# Autodesk Inventor assembly: fullbox
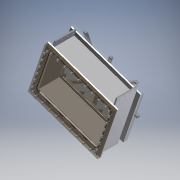
[picture p0: Inventor's stored thumbnail of the model, 180x180]
Saved by Autodesk Inventor 2017 (Build 210142000, 142)
## iProperties
Created: 2017-08-02
Part Number: fullbox
Document SubType Name: Assembly
Designer: Kai
Author: Kai
## Documents named in this file (14)
- D:\robosub\fullbox.iam
- C:\Users\Kai\Documents\Sub_stuff\2018sub\box2.0\longsides.ipt
- C:\Users\Kai\Documents\Sub_stuff\2018sub\box2.0\shortsides.ipt
- C:\Users\Kai\Documents\Sub_stuff\2018sub\box2.0\smallgasketback.ipt
- C:\Users\Kai\Downloads\91292A137_TYPE 18-8 SS SOCKET HEAD CAP SCREW.ipt
- C:\Users\Kai\Documents\Sub_stuff\2018sub\box2.0\top.ipt
- C:\Users\Kai\Documents\Sub_stuff\2018sub\box2.0\toppoly.ipt
- C:\Users\Kai\Documents\Sub_stuff\2018sub\box2.0\bottom3.ipt
- C:\Users\Kai\Documents\Sub_stuff\2018sub\box2.0\alumbottom3.ipt
- C:\Users\Kai\Documents\Sub_stuff\2018sub\box2.0\lock\pin holder.ipt
- C:\Users\Kai\Documents\Sub_stuff\2018sub\box2.0\lock\pins.ipt
- C:\Users\Kai\Downloads\91292A134_TYPE 18-8 SS SOCKET HEAD CAP SCREW.ipt
- C:\Users\Kai\Documents\Sub_stuff\2018sub\box2.0\lid guide.ipt
- C:\Users\Kai\Downloads\99397A074_METRIC THREAD-FORMING SCREW FOR PLASTICS.ipt
## Components (65 placed, 13 different names)
1. longsides:1 — Mate:6, Flush:8
2. longsides:2 — Mate:3, Mate:106, Mate:107, Mate:108, Mate:109, Flush:3
3. shortsides:1 — Mate:3, Mate:106, Mate:108, Flush:9, Mate:116
4. shortsides:2 — Mate:6, Mate:107, Mate:109, Mate:111, Mate:112
5. smallgasketback:1 — Mate:117, Mate:118
6. top:1 — Mate:111, Mate:112, Flush:3, Mate:113, Mate:114, Mate:115, Flush:4, Flush:5, Mate:213, Mate:214
7. smallgasketback:2 — Mate:113, Mate:114
8. toppoly:1 — Mate:115, Flush:4, Flush:5, Mate:193, Flush:10, Flush:11, Mate:212
9. bottom3:1 — Mate:119, Mate:120, Mate:121, Mate:122, Mate:123, Mate:124, Mate:125, Mate:126, Mate:127, Mate:128, Mate:129, Mate:130, Mate:131, Mate:132, Mate:133, Mate:134, Mate:135, Mate:136, Mate:137, Mate:138, Mate:139, Mate:140, Mate:141, Mate:142, Mate:143, Mate:144, Mate:145, Mate:146, Mate:147, Mate:148, Mate:149, Mate:150, Mate:151, Mate:152, Mate:153, Mate:154, Mate:155, Mate:156, Mate:157, Mate:158, Mate:159, Mate:160, Mate:161, Mate:162, Mate:163, Mate:164, Mate:165, Mate:166, Mate:167, Mate:168, Mate:169, Mate:170, Mate:171, Mate:172, Mate:173, Mate:174, Mate:175, Mate:176, Mate:177, Mate:178, Mate:179, Mate:180, Mate:181, Mate:182, Mate:183, Mate:184, Mate:185, Mate:186, Mate:187, Mate:188, Mate:189
10. alumbottom3:1 — Flush:8, Flush:9, Mate:116, Mate:117, Mate:118, Mate:119, Mate:120, Mate:121
11. 91292A137_TYPE 18-8 SS SOCKET HEAD CAP SCREW:1 — Mate:123, Mate:188
12. 91292A137_TYPE 18-8 SS SOCKET HEAD CAP SCREW:2 — Mate:124, Mate:189
13. 91292A137_TYPE 18-8 SS SOCKET HEAD CAP SCREW:3 — Mate:125, Mate:158
14. 91292A137_TYPE 18-8 SS SOCKET HEAD CAP SCREW:4 — Mate:126, Mate:157
15. 91292A137_TYPE 18-8 SS SOCKET HEAD CAP SCREW:5 — Mate:127, Mate:156
16. 91292A137_TYPE 18-8 SS SOCKET HEAD CAP SCREW:6 — Mate:128, Mate:159
17. 91292A137_TYPE 18-8 SS SOCKET HEAD CAP SCREW:7 — Mate:129, Mate:160
18. 91292A137_TYPE 18-8 SS SOCKET HEAD CAP SCREW:8 — Mate:130, Mate:161
19. 91292A137_TYPE 18-8 SS SOCKET HEAD CAP SCREW:9 — Mate:131, Mate:162
20. 91292A137_TYPE 18-8 SS SOCKET HEAD CAP SCREW:10 — Mate:132, Mate:163
21. 91292A137_TYPE 18-8 SS SOCKET HEAD CAP SCREW:11 — Mate:133, Mate:164
22. 91292A137_TYPE 18-8 SS SOCKET HEAD CAP SCREW:12 — Mate:134, Mate:165
23. 91292A137_TYPE 18-8 SS SOCKET HEAD CAP SCREW:13 — Mate:135, Mate:166
24. 91292A137_TYPE 18-8 SS SOCKET HEAD CAP SCREW:14 — Mate:136, Mate:167
25. 91292A137_TYPE 18-8 SS SOCKET HEAD CAP SCREW:15 — Mate:137, Mate:168
26. 91292A137_TYPE 18-8 SS SOCKET HEAD CAP SCREW:16 — Mate:138, Mate:169
27. 91292A137_TYPE 18-8 SS SOCKET HEAD CAP SCREW:17 — Mate:139, Mate:170
28. 91292A137_TYPE 18-8 SS SOCKET HEAD CAP SCREW:18 — Mate:140, Mate:171
29. 91292A137_TYPE 18-8 SS SOCKET HEAD CAP SCREW:19 — Mate:141, Mate:172
30. 91292A137_TYPE 18-8 SS SOCKET HEAD CAP SCREW:20 — Mate:142, Mate:173
31. 91292A137_TYPE 18-8 SS SOCKET HEAD CAP SCREW:21 — Mate:144, Mate:175
32. 91292A137_TYPE 18-8 SS SOCKET HEAD CAP SCREW:22 — Mate:143, Mate:174
33. 91292A137_TYPE 18-8 SS SOCKET HEAD CAP SCREW:23 — Mate:145, Mate:176
34. 91292A137_TYPE 18-8 SS SOCKET HEAD CAP SCREW:24 — Mate:147, Mate:178
35. 91292A137_TYPE 18-8 SS SOCKET HEAD CAP SCREW:25 — Mate:148, Mate:179
36. 91292A137_TYPE 18-8 SS SOCKET HEAD CAP SCREW:26 — Mate:149, Mate:180
37. 91292A137_TYPE 18-8 SS SOCKET HEAD CAP SCREW:27 — Mate:150, Mate:181
38. 91292A137_TYPE 18-8 SS SOCKET HEAD CAP SCREW:28 — Mate:151, Mate:182
39. 91292A137_TYPE 18-8 SS SOCKET HEAD CAP SCREW:29 — Mate:152, Mate:183
40. 91292A137_TYPE 18-8 SS SOCKET HEAD CAP SCREW:30 — Mate:153, Mate:184
41. 91292A137_TYPE 18-8 SS SOCKET HEAD CAP SCREW:31 — Mate:154, Mate:185
42. 91292A137_TYPE 18-8 SS SOCKET HEAD CAP SCREW:32 — Mate:155, Mate:186
43. 91292A137_TYPE 18-8 SS SOCKET HEAD CAP SCREW:33 — Mate:146, Mate:177
44. 91292A137_TYPE 18-8 SS SOCKET HEAD CAP SCREW:34 — Mate:122, Mate:187
45. pin holder:1 — Mate:194, Mate:195
46. pins:1 — Mate:193, Mate:194, Mate:195, Flush:10, Flush:11, Mate:196, Mate:197, Mate:198, Mate:199, Mate:200, Mate:201, Mate:202, Mate:203, Mate:204, Mate:205, Mate:206, Mate:207, Mate:208, Mate:209, Mate:210, Mate:211
47. 91292A134_TYPE 18-8 SS SOCKET HEAD CAP SCREW:1 — Mate:199, Mate:208
48. 91292A134_TYPE 18-8 SS SOCKET HEAD CAP SCREW:2 — Mate:201, Mate:205
49. 91292A134_TYPE 18-8 SS SOCKET HEAD CAP SCREW:3 — Mate:200, Mate:207
50. 91292A134_TYPE 18-8 SS SOCKET HEAD CAP SCREW:4 — Mate:202, Mate:211
51. 91292A134_TYPE 18-8 SS SOCKET HEAD CAP SCREW:5 — Mate:197, Mate:209
52. 91292A134_TYPE 18-8 SS SOCKET HEAD CAP SCREW:6 — Mate:196, Mate:204
53. 91292A134_TYPE 18-8 SS SOCKET HEAD CAP SCREW:7 — Mate:198, Mate:210
54. 91292A134_TYPE 18-8 SS SOCKET HEAD CAP SCREW:8 — Mate:203, Mate:206
55. lid guide:1 — Mate:212, Mate:213, Mate:214, Mate:215, Mate:216, Mate:217, Mate:218, Mate:219, Mate:220, Mate:221, Mate:222, Mate:223, Mate:224, Mate:225, Mate:226, Mate:227, Mate:228, Mate:229, Mate:230, Mate:231, Mate:232, Mate:233, Mate:234
56. 99397A074_METRIC THREAD-FORMING SCREW FOR PLASTICS:1 — Mate:224, Mate:226
57. 99397A074_METRIC THREAD-FORMING SCREW FOR PLASTICS:2 — Mate:215, Mate:231
58. 99397A074_METRIC THREAD-FORMING SCREW FOR PLASTICS:3 — Mate:221, Mate:228
59. 99397A074_METRIC THREAD-FORMING SCREW FOR PLASTICS:4 — Mate:222, Mate:227
60. 99397A074_METRIC THREAD-FORMING SCREW FOR PLASTICS:5 — Mate:217, Mate:230
61. 99397A074_METRIC THREAD-FORMING SCREW FOR PLASTICS:6 — Mate:216, Mate:232
62. 99397A074_METRIC THREAD-FORMING SCREW FOR PLASTICS:7 — Mate:223, Mate:225
63. 99397A074_METRIC THREAD-FORMING SCREW FOR PLASTICS:8 — Mate:219, Mate:229
64. 99397A074_METRIC THREAD-FORMING SCREW FOR PLASTICS:9 — Mate:218, Mate:233
65. 99397A074_METRIC THREAD-FORMING SCREW FOR PLASTICS:10 — Mate:220, Mate:234
## Relationships (134: Mate 127, Flush 7)
- Mate:3: longsides:2 ↔ shortsides:1
- Mate:6: longsides:1 ↔ shortsides:2
- Mate:106: longsides:2 ↔ shortsides:1
- Mate:107: longsides:2 ↔ shortsides:2
- Mate:108: longsides:2 ↔ shortsides:1
- Mate:109: longsides:2 ↔ shortsides:2
- Mate:111: shortsides:2 ↔ top:1
- Mate:112 (304.8 mm): shortsides:2 ↔ top:1
- Flush:3 (-19.05 mm): longsides:2 ↔ top:1
- Mate:113: top:1 ↔ smallgasketback:2
- Mate:114: top:1 ↔ smallgasketback:2
- Mate:115: top:1 ↔ toppoly:1
- Flush:4: top:1 ↔ toppoly:1
- Flush:5: top:1 ↔ toppoly:1
- Flush:8: longsides:1 ↔ alumbottom3:1
- Flush:9: shortsides:1 ↔ alumbottom3:1
- Mate:116: shortsides:1 ↔ alumbottom3:1
- Mate:117: smallgasketback:1 ↔ alumbottom3:1
- Mate:118: smallgasketback:1 ↔ alumbottom3:1
- Mate:119: bottom3:1 ↔ alumbottom3:1
- Mate:120: bottom3:1 ↔ alumbottom3:1
- Mate:121: bottom3:1 ↔ alumbottom3:1
- Mate:122: bottom3:1 ↔ 91292A137_TYPE 18-8 SS SOCKET HEAD CAP SCREW:34
- Mate:123: bottom3:1 ↔ 91292A137_TYPE 18-8 SS SOCKET HEAD CAP SCREW:1
- Mate:124: bottom3:1 ↔ 91292A137_TYPE 18-8 SS SOCKET HEAD CAP SCREW:2
- Mate:125: bottom3:1 ↔ 91292A137_TYPE 18-8 SS SOCKET HEAD CAP SCREW:3
- Mate:126: bottom3:1 ↔ 91292A137_TYPE 18-8 SS SOCKET HEAD CAP SCREW:4
- Mate:127: bottom3:1 ↔ 91292A137_TYPE 18-8 SS SOCKET HEAD CAP SCREW:5
- Mate:128: bottom3:1 ↔ 91292A137_TYPE 18-8 SS SOCKET HEAD CAP SCREW:6
- Mate:129: bottom3:1 ↔ 91292A137_TYPE 18-8 SS SOCKET HEAD CAP SCREW:7
- Mate:130: bottom3:1 ↔ 91292A137_TYPE 18-8 SS SOCKET HEAD CAP SCREW:8
- Mate:131: bottom3:1 ↔ 91292A137_TYPE 18-8 SS SOCKET HEAD CAP SCREW:9
- Mate:132: bottom3:1 ↔ 91292A137_TYPE 18-8 SS SOCKET HEAD CAP SCREW:10
- Mate:133: bottom3:1 ↔ 91292A137_TYPE 18-8 SS SOCKET HEAD CAP SCREW:11
- Mate:134: bottom3:1 ↔ 91292A137_TYPE 18-8 SS SOCKET HEAD CAP SCREW:12
- Mate:135: bottom3:1 ↔ 91292A137_TYPE 18-8 SS SOCKET HEAD CAP SCREW:13
- Mate:136: bottom3:1 ↔ 91292A137_TYPE 18-8 SS SOCKET HEAD CAP SCREW:14
- Mate:137: bottom3:1 ↔ 91292A137_TYPE 18-8 SS SOCKET HEAD CAP SCREW:15
- Mate:138: bottom3:1 ↔ 91292A137_TYPE 18-8 SS SOCKET HEAD CAP SCREW:16
- Mate:139: bottom3:1 ↔ 91292A137_TYPE 18-8 SS SOCKET HEAD CAP SCREW:17
- Mate:140: bottom3:1 ↔ 91292A137_TYPE 18-8 SS SOCKET HEAD CAP SCREW:18
- Mate:141: bottom3:1 ↔ 91292A137_TYPE 18-8 SS SOCKET HEAD CAP SCREW:19
- Mate:142: bottom3:1 ↔ 91292A137_TYPE 18-8 SS SOCKET HEAD CAP SCREW:20
- Mate:143: bottom3:1 ↔ 91292A137_TYPE 18-8 SS SOCKET HEAD CAP SCREW:22
- Mate:144: bottom3:1 ↔ 91292A137_TYPE 18-8 SS SOCKET HEAD CAP SCREW:21
- Mate:145: bottom3:1 ↔ 91292A137_TYPE 18-8 SS SOCKET HEAD CAP SCREW:23
- Mate:146: bottom3:1 ↔ 91292A137_TYPE 18-8 SS SOCKET HEAD CAP SCREW:33
- Mate:147: bottom3:1 ↔ 91292A137_TYPE 18-8 SS SOCKET HEAD CAP SCREW:24
- Mate:148: bottom3:1 ↔ 91292A137_TYPE 18-8 SS SOCKET HEAD CAP SCREW:25
- Mate:149: bottom3:1 ↔ 91292A137_TYPE 18-8 SS SOCKET HEAD CAP SCREW:26
- Mate:150: bottom3:1 ↔ 91292A137_TYPE 18-8 SS SOCKET HEAD CAP SCREW:27
- Mate:151: bottom3:1 ↔ 91292A137_TYPE 18-8 SS SOCKET HEAD CAP SCREW:28
- Mate:152: bottom3:1 ↔ 91292A137_TYPE 18-8 SS SOCKET HEAD CAP SCREW:29
- Mate:153: bottom3:1 ↔ 91292A137_TYPE 18-8 SS SOCKET HEAD CAP SCREW:30
- Mate:154: bottom3:1 ↔ 91292A137_TYPE 18-8 SS SOCKET HEAD CAP SCREW:31
- Mate:155: bottom3:1 ↔ 91292A137_TYPE 18-8 SS SOCKET HEAD CAP SCREW:32
- Mate:156: bottom3:1 ↔ 91292A137_TYPE 18-8 SS SOCKET HEAD CAP SCREW:5
- Mate:157: bottom3:1 ↔ 91292A137_TYPE 18-8 SS SOCKET HEAD CAP SCREW:4
- Mate:158: bottom3:1 ↔ 91292A137_TYPE 18-8 SS SOCKET HEAD CAP SCREW:3
- Mate:159: bottom3:1 ↔ 91292A137_TYPE 18-8 SS SOCKET HEAD CAP SCREW:6
- Mate:160: bottom3:1 ↔ 91292A137_TYPE 18-8 SS SOCKET HEAD CAP SCREW:7
- Mate:161: bottom3:1 ↔ 91292A137_TYPE 18-8 SS SOCKET HEAD CAP SCREW:8
- Mate:162: bottom3:1 ↔ 91292A137_TYPE 18-8 SS SOCKET HEAD CAP SCREW:9
- Mate:163: bottom3:1 ↔ 91292A137_TYPE 18-8 SS SOCKET HEAD CAP SCREW:10
- Mate:164: bottom3:1 ↔ 91292A137_TYPE 18-8 SS SOCKET HEAD CAP SCREW:11
- Mate:165: bottom3:1 ↔ 91292A137_TYPE 18-8 SS SOCKET HEAD CAP SCREW:12
- Mate:166: bottom3:1 ↔ 91292A137_TYPE 18-8 SS SOCKET HEAD CAP SCREW:13
- Mate:167: bottom3:1 ↔ 91292A137_TYPE 18-8 SS SOCKET HEAD CAP SCREW:14
- Mate:168: bottom3:1 ↔ 91292A137_TYPE 18-8 SS SOCKET HEAD CAP SCREW:15
- Mate:169: bottom3:1 ↔ 91292A137_TYPE 18-8 SS SOCKET HEAD CAP SCREW:16
- Mate:170: bottom3:1 ↔ 91292A137_TYPE 18-8 SS SOCKET HEAD CAP SCREW:17
- Mate:171: bottom3:1 ↔ 91292A137_TYPE 18-8 SS SOCKET HEAD CAP SCREW:18
- Mate:172: bottom3:1 ↔ 91292A137_TYPE 18-8 SS SOCKET HEAD CAP SCREW:19
- Mate:173: bottom3:1 ↔ 91292A137_TYPE 18-8 SS SOCKET HEAD CAP SCREW:20
- Mate:174: bottom3:1 ↔ 91292A137_TYPE 18-8 SS SOCKET HEAD CAP SCREW:22
- Mate:175: bottom3:1 ↔ 91292A137_TYPE 18-8 SS SOCKET HEAD CAP SCREW:21
- Mate:176: bottom3:1 ↔ 91292A137_TYPE 18-8 SS SOCKET HEAD CAP SCREW:23
- Mate:177: bottom3:1 ↔ 91292A137_TYPE 18-8 SS SOCKET HEAD CAP SCREW:33
- Mate:178: bottom3:1 ↔ 91292A137_TYPE 18-8 SS SOCKET HEAD CAP SCREW:24
- Mate:179: bottom3:1 ↔ 91292A137_TYPE 18-8 SS SOCKET HEAD CAP SCREW:25
- Mate:180: bottom3:1 ↔ 91292A137_TYPE 18-8 SS SOCKET HEAD CAP SCREW:26
- Mate:181: bottom3:1 ↔ 91292A137_TYPE 18-8 SS SOCKET HEAD CAP SCREW:27
- Mate:182: bottom3:1 ↔ 91292A137_TYPE 18-8 SS SOCKET HEAD CAP SCREW:28
- Mate:183: bottom3:1 ↔ 91292A137_TYPE 18-8 SS SOCKET HEAD CAP SCREW:29
- Mate:184: bottom3:1 ↔ 91292A137_TYPE 18-8 SS SOCKET HEAD CAP SCREW:30
- Mate:185: bottom3:1 ↔ 91292A137_TYPE 18-8 SS SOCKET HEAD CAP SCREW:31
- Mate:186: bottom3:1 ↔ 91292A137_TYPE 18-8 SS SOCKET HEAD CAP SCREW:32
- Mate:187: bottom3:1 ↔ 91292A137_TYPE 18-8 SS SOCKET HEAD CAP SCREW:34
- Mate:188: bottom3:1 ↔ 91292A137_TYPE 18-8 SS SOCKET HEAD CAP SCREW:1
- Mate:189: bottom3:1 ↔ 91292A137_TYPE 18-8 SS SOCKET HEAD CAP SCREW:2
- Mate:193: toppoly:1 ↔ pins:1
- Mate:194: pin holder:1 ↔ pins:1
- Mate:195: pin holder:1 ↔ pins:1
- Flush:10 (-6.35 mm): toppoly:1 ↔ pins:1
- Flush:11 (-6.35 mm): toppoly:1 ↔ pins:1
- Mate:196: pins:1 ↔ 91292A134_TYPE 18-8 SS SOCKET HEAD CAP SCREW:6
- Mate:197: pins:1 ↔ 91292A134_TYPE 18-8 SS SOCKET HEAD CAP SCREW:5
- Mate:198: pins:1 ↔ 91292A134_TYPE 18-8 SS SOCKET HEAD CAP SCREW:7
- Mate:199: pins:1 ↔ 91292A134_TYPE 18-8 SS SOCKET HEAD CAP SCREW:1
- Mate:200: pins:1 ↔ 91292A134_TYPE 18-8 SS SOCKET HEAD CAP SCREW:3
- Mate:201: pins:1 ↔ 91292A134_TYPE 18-8 SS SOCKET HEAD CAP SCREW:2
- Mate:202: pins:1 ↔ 91292A134_TYPE 18-8 SS SOCKET HEAD CAP SCREW:4
- Mate:203: pins:1 ↔ 91292A134_TYPE 18-8 SS SOCKET HEAD CAP SCREW:8
- Mate:204: pins:1 ↔ 91292A134_TYPE 18-8 SS SOCKET HEAD CAP SCREW:6
- Mate:205: pins:1 ↔ 91292A134_TYPE 18-8 SS SOCKET HEAD CAP SCREW:2
- Mate:206: pins:1 ↔ 91292A134_TYPE 18-8 SS SOCKET HEAD CAP SCREW:8
- Mate:207: pins:1 ↔ 91292A134_TYPE 18-8 SS SOCKET HEAD CAP SCREW:3
- Mate:208: pins:1 ↔ 91292A134_TYPE 18-8 SS SOCKET HEAD CAP SCREW:1
- Mate:209: pins:1 ↔ 91292A134_TYPE 18-8 SS SOCKET HEAD CAP SCREW:5
- Mate:210: pins:1 ↔ 91292A134_TYPE 18-8 SS SOCKET HEAD CAP SCREW:7
- Mate:211: pins:1 ↔ 91292A134_TYPE 18-8 SS SOCKET HEAD CAP SCREW:4
- Mate:212: toppoly:1 ↔ lid guide:1
- Mate:213: top:1 ↔ lid guide:1
- Mate:214: top:1 ↔ lid guide:1
- Mate:215: lid guide:1 ↔ 99397A074_METRIC THREAD-FORMING SCREW FOR PLASTICS:2
- Mate:216: lid guide:1 ↔ 99397A074_METRIC THREAD-FORMING SCREW FOR PLASTICS:6
- Mate:217: lid guide:1 ↔ 99397A074_METRIC THREAD-FORMING SCREW FOR PLASTICS:5
- Mate:218: lid guide:1 ↔ 99397A074_METRIC THREAD-FORMING SCREW FOR PLASTICS:9
- Mate:219: lid guide:1 ↔ 99397A074_METRIC THREAD-FORMING SCREW FOR PLASTICS:8
- Mate:220: lid guide:1 ↔ 99397A074_METRIC THREAD-FORMING SCREW FOR PLASTICS:10
- Mate:221: lid guide:1 ↔ 99397A074_METRIC THREAD-FORMING SCREW FOR PLASTICS:3
- Mate:222: lid guide:1 ↔ 99397A074_METRIC THREAD-FORMING SCREW FOR PLASTICS:4
- Mate:223: lid guide:1 ↔ 99397A074_METRIC THREAD-FORMING SCREW FOR PLASTICS:7
- Mate:224: lid guide:1 ↔ 99397A074_METRIC THREAD-FORMING SCREW FOR PLASTICS:1
- Mate:225: lid guide:1 ↔ 99397A074_METRIC THREAD-FORMING SCREW FOR PLASTICS:7
- Mate:226: lid guide:1 ↔ 99397A074_METRIC THREAD-FORMING SCREW FOR PLASTICS:1
- Mate:227: lid guide:1 ↔ 99397A074_METRIC THREAD-FORMING SCREW FOR PLASTICS:4
- Mate:228: lid guide:1 ↔ 99397A074_METRIC THREAD-FORMING SCREW FOR PLASTICS:3
- Mate:229: lid guide:1 ↔ 99397A074_METRIC THREAD-FORMING SCREW FOR PLASTICS:8
- Mate:230: lid guide:1 ↔ 99397A074_METRIC THREAD-FORMING SCREW FOR PLASTICS:5
- Mate:231: lid guide:1 ↔ 99397A074_METRIC THREAD-FORMING SCREW FOR PLASTICS:2
- Mate:232: lid guide:1 ↔ 99397A074_METRIC THREAD-FORMING SCREW FOR PLASTICS:6
- Mate:233: lid guide:1 ↔ 99397A074_METRIC THREAD-FORMING SCREW FOR PLASTICS:9
- Mate:234: lid guide:1 ↔ 99397A074_METRIC THREAD-FORMING SCREW FOR PLASTICS:10
